# Autodesk Inventor assembly: 8100_Tx_Filter_Stage1_Layout_v1
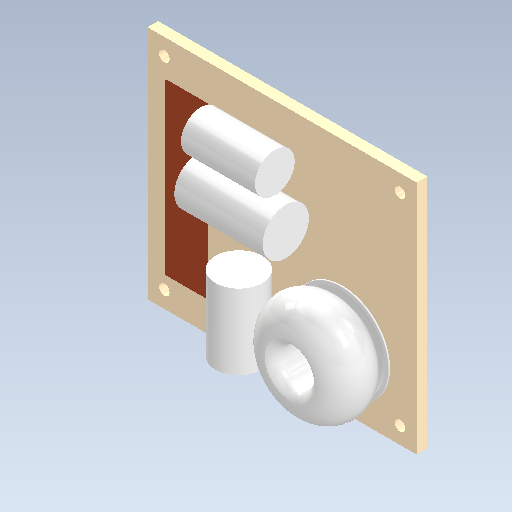
[picture p0: Inventor's stored thumbnail of the model, 512x512]
Saved by Autodesk Inventor 2021 (Build 250183000, 183)
## iProperties
Created: 2021-04-07
Part Number: 8100_Tx_Filter_Stage1_Layout_v1
Document SubType Name: Assembly
Designer: Barksdale
Author: Barksdale
## Documents named in this file (8)
- C:\Users\Barksdale\Dropbox (MIT)\MPI Group Folder\MPS\Inventor_Parts and MPSv2 all folder\MPSV2\Tx Filter\8100_Tx_Filter_Stage1_Layout_v1.iam
- C:\Users\Barksdale\Dropbox (MIT)\MPI Group Folder\MPS\Inventor_Parts and MPSv2 all folder\MPSV2\Tx Filter\8000_132uH_DCore_2layer_Tx_Filter_MPSv2_v1.ipt
- C:\Users\Barksdale\Dropbox (MIT)\MPI Group Folder\MPS\Inventor_Parts and MPSv2 all folder\MPSV2\Tx Filter\8002_base_132uH_DCore_2layer_Tx_Filter_MPSv2_v1.ipt
- C:\Users\Barksdale\Dropbox (MIT)\MPI Group Folder\MPS\Inventor_Parts and MPSv2 all folder\MPSV2\Tx Filter\8010_2uF_Tx_Capacitor_v1.ipt
- C:\Users\Barksdale\Dropbox (MIT)\MPI Group Folder\MPS\Inventor_Parts and MPSv2 all folder\MPSV2\Tx Filter\8011_1uF_Tx_Capacitor_v1.ipt
- C:\Users\Barksdale\Dropbox (MIT)\MPI Group Folder\MPS\Inventor_Parts and MPSv2 all folder\MPSV2\Tx Filter\8012_560nF_Tx_Capacitor_v1.ipt
- C:\Users\Barksdale\Dropbox (MIT)\MPI Group Folder\MPS\Inventor_Parts and MPSv2 all folder\MPSV2\Tx Filter\8020_Base_Tx_Filter_v1.ipt
- C:\Users\Barksdale\Dropbox (MIT)\MPI Group Folder\MPS\Inventor_Parts and MPSv2 all folder\MPSV2\Tx Filter\8005_Cu_groundplane_Tx_Filter_Stage1_MPSv2_v1.ipt
## Components (7 placed, 7 different names)
1. 8000_132uH_DCore_2layer_Tx_Filter_MPSv2_v1:1 — Mate:2, Mate:3
2. 8002_base_132uH_DCore_2layer_Tx_Filter_MPSv2_v1:1 — Mate:1, Mate:2, Mate:3
3. 8010_2uF_Tx_Capacitor_v1:1 — Tangent:1
4. 8011_1uF_Tx_Capacitor_v1:1 — Tangent:3, Angle:2, Flush:1
5. 8012_560nF_Tx_Capacitor_v1:1 — Tangent:2, Flush:1
6. 8020_Base_Tx_Filter_v1:1 — Mate:1, Tangent:1, Tangent:2, Tangent:3, Mate:4, Angle:1, Angle:2
7. 8005_Cu_groundplane_Tx_Filter_Stage1_MPSv2_v1:1 — Mate:4, Angle:1
## Relationships (10: Mate 4, Tangent 3, Angle 2, Flush 1)
- Mate:1: 8002_base_132uH_DCore_2layer_Tx_Filter_MPSv2_v1:1 ↔ 8020_Base_Tx_Filter_v1:1
- Mate:2: 8000_132uH_DCore_2layer_Tx_Filter_MPSv2_v1:1 ↔ 8002_base_132uH_DCore_2layer_Tx_Filter_MPSv2_v1:1
- Mate:3: 8000_132uH_DCore_2layer_Tx_Filter_MPSv2_v1:1 ↔ 8002_base_132uH_DCore_2layer_Tx_Filter_MPSv2_v1:1
- Tangent:1: 8010_2uF_Tx_Capacitor_v1:1 ↔ 8020_Base_Tx_Filter_v1:1
- Tangent:2: 8012_560nF_Tx_Capacitor_v1:1 ↔ 8020_Base_Tx_Filter_v1:1
- Tangent:3: 8011_1uF_Tx_Capacitor_v1:1 ↔ 8020_Base_Tx_Filter_v1:1
- Mate:4: 8020_Base_Tx_Filter_v1:1 ↔ 8005_Cu_groundplane_Tx_Filter_Stage1_MPSv2_v1:1
- Angle:1 (0 deg): 8020_Base_Tx_Filter_v1:1 ↔ 8005_Cu_groundplane_Tx_Filter_Stage1_MPSv2_v1:1
- Angle:2 (0 deg): 8011_1uF_Tx_Capacitor_v1:1 ↔ 8020_Base_Tx_Filter_v1:1
- Flush:1: 8011_1uF_Tx_Capacitor_v1:1 ↔ 8012_560nF_Tx_Capacitor_v1:1
